# Autodesk Inventor assembly: AVADemo_SlidingDoor
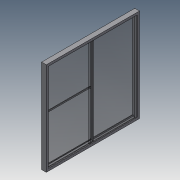
[picture p0: Inventor's stored thumbnail of the model, 180x180]
Saved by Autodesk Inventor 2018.3 (Build 223284000, 284)
## iProperties
RuleStatus: InUse
Created: 2019-11-06
Part Number: AVADemo_SlidingDoor
Document SubType Name: Assembly
Designer: MattBussey
Author: MattBussey
## Documents named in this file (3)
- C:\AVAInvAPI\Workspace\Output\AVADemo_SlidingDoor.iam
- C:\AVAInvAPI\Workspace\Output\AVADemo_SlidingDoorFrame.ipt
- C:\AVAInvAPI\Workspace\Output\AVADemo_SlidingDoorPanel.ipt
## Components (2 placed, 2 different names)
1. AVADemo_SlidingDoorFrame:1 — Mate:1, FloorMate, MateLeft, MateInterior, MateRight, MateExterior
2. AVADemo_SlidingDoorPanel:1 — FloorMate, MateLeft, MateInterior, MateRight, MateExterior
## Relationships (6: Mate 6)
- Mate:1: AVADemo_SlidingDoorFrame:1
- FloorMate [Mate]: AVADemo_SlidingDoorFrame:1 ↔ AVADemo_SlidingDoorPanel:1
- MateLeft: AVADemo_SlidingDoorFrame:1 ↔ AVADemo_SlidingDoorPanel:1
- MateInterior: AVADemo_SlidingDoorFrame:1 ↔ AVADemo_SlidingDoorPanel:1
- MateRight: AVADemo_SlidingDoorFrame:1 ↔ AVADemo_SlidingDoorPanel:1
- MateExterior: AVADemo_SlidingDoorFrame:1 ↔ AVADemo_SlidingDoorPanel:1
## Named parameters: Width = 2032 mm, Depth = 101.6 mm, Height = 2032 mm
